# Autodesk Inventor assembly: Robot_Assembly2
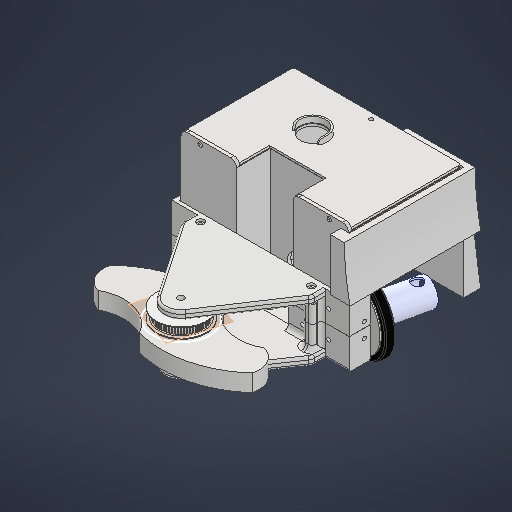
[picture p0: Inventor's stored thumbnail of the model, 512x512]
Saved by Autodesk Inventor 2026.2 (Build 302298000, 298)
## iProperties
Created: 2026-02-14
Part Number: Robot_Assembly2
Document SubType Name: Assembly
Designer: chigg
Author: chigg
## Documents named in this file (10)
- C:\Users\chigg\Robot_Spring_Semester\Robot_Model\Robot_Assembly2.iam
- C:\Users\chigg\Robot_Spring_Semester\Robot_Model\02)_Chassis V5 - Horizotal, Medium.ipt
- C:\Users\chigg\Robot_Spring_Semester\Robot_Model\Wheel And Motor.iam
- C:\Users\chigg\Robot_Spring_Semester\Robot_Model\Servo.ipt
- C:\Users\chigg\Robot_Spring_Semester\Robot_Model\03)_Base Lid V5 - Horizontal.ipt
- C:\Users\chigg\Robot_Spring_Semester\Robot_Model\11)_Weapon Mount V5 - Horizontal, Top Half.ipt
- C:\Users\chigg\Robot_Spring_Semester\Robot_Model\10)_Weapon Mount V5 - Horizontal, Bottom Half.ipt
- C:\Users\chigg\Robot_Spring_Semester\Robot_Model\Servo Horn.ipt
- C:\Users\chigg\Robot_Spring_Semester\Robot_Model\07)_Weapon Assembly V5 - Horizotal Spinner.iam
- C:\Users\chigg\Robot_Spring_Semester\Robot_Model\04)_Side Armor V5 - Left, Horizontal.ipt
## Components (12 placed, 9 different names)
1. 02)_Chassis V5 - Horizotal, Medium:1 — Mate:1, Flush:1, Mate:2, Flush:2, Mate:3, Mate:4, Mate:5, Mate:6, Insert:3, Insert:4, Mate:8
2. Wheel And Motor:1 [sub-assembly] — Insert:1
3. Servo:1 — Mate:1, Flush:1, Rotational:1, Mate:5
4. Servo:2 — Mate:2, Flush:2, Rotational:2, Mate:6
5. 03)_Base Lid V5 - Horizontal:1 — Mate:3, Mate:4, Flush:3
6. 11)_Weapon Mount V5 - Horizontal, Top Half:1 — Insert:3, Mate:7
7. 10)_Weapon Mount V5 - Horizontal, Bottom Half:1 — Insert:4, Mate:7, Insert:5
8. Servo Horn:1 — Rotational:1, Insert:1
9. Servo Horn:2 — Rotational:2, Insert:2
10. Wheel And Motor:2 [sub-assembly] — Insert:2
11. 07)_Weapon Assembly V5 - Horizotal Spinner:1 [sub-assembly] — Insert:5
12. 04)_Side Armor V5 - Left, Horizontal:1 — Mate:8, Flush:3
## Relationships (18: Mate 8, Insert 5, Flush 3, RevoluteJoint 2)
- Mate:1: 02)_Chassis V5 - Horizotal, Medium:1 ↔ Servo:1
- Flush:1: 02)_Chassis V5 - Horizotal, Medium:1 ↔ Servo:1
- Mate:2: 02)_Chassis V5 - Horizotal, Medium:1 ↔ Servo:2
- Flush:2: 02)_Chassis V5 - Horizotal, Medium:1 ↔ Servo:2
- Mate:3: 02)_Chassis V5 - Horizotal, Medium:1 ↔ 03)_Base Lid V5 - Horizontal:1
- Mate:4: 02)_Chassis V5 - Horizotal, Medium:1 ↔ 03)_Base Lid V5 - Horizontal:1
- Rotational:1 [RevoluteJoint] (-4.5 mm): Servo:1 ↔ Servo Horn:1
- Insert:1: Wheel And Motor:1 ↔ Servo Horn:1
- Mate:5: 02)_Chassis V5 - Horizotal, Medium:1 ↔ Servo:1
- Rotational:2 [RevoluteJoint] (-4.5 mm): Servo:2 ↔ Servo Horn:2
- Mate:6: 02)_Chassis V5 - Horizotal, Medium:1 ↔ Servo:2
- Insert:2: Servo Horn:2 ↔ Wheel And Motor:2
- Insert:3: 02)_Chassis V5 - Horizotal, Medium:1 ↔ 11)_Weapon Mount V5 - Horizontal, Top Half:1
- Insert:4: 02)_Chassis V5 - Horizotal, Medium:1 ↔ 10)_Weapon Mount V5 - Horizontal, Bottom Half:1
- Mate:7: 11)_Weapon Mount V5 - Horizontal, Top Half:1 ↔ 10)_Weapon Mount V5 - Horizontal, Bottom Half:1
- Insert:5: 10)_Weapon Mount V5 - Horizontal, Bottom Half:1 ↔ 07)_Weapon Assembly V5 - Horizotal Spinner:1
- Mate:8: 02)_Chassis V5 - Horizotal, Medium:1 ↔ 04)_Side Armor V5 - Left, Horizontal:1
- Flush:3 (2 mm): 03)_Base Lid V5 - Horizontal:1 ↔ 04)_Side Armor V5 - Left, Horizontal:1
